# Autodesk Inventor assembly: Complete Device
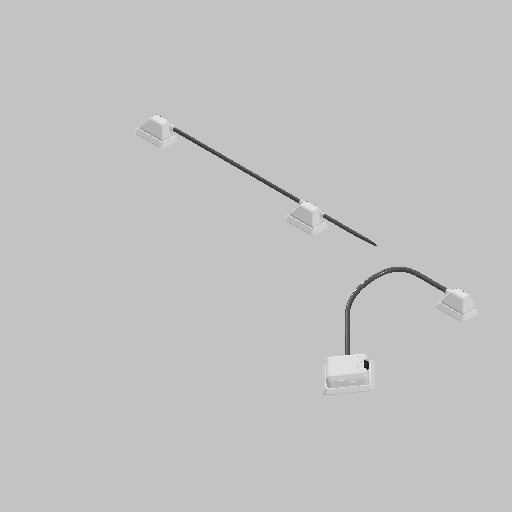
[picture p0: Inventor's stored thumbnail of the model, 512x512]
Saved by Autodesk Inventor 2025.2 (Build 292293000, 293)
## iProperties
Created: 2024-11-20
Part Number: Complete Device
Document SubType Name: Assembly
Designer: tills
Author: tills
## Documents named in this file (8)
- C:\Users\matss\Documents\.Studium\Health_Device\CAD\Wearable-Health-Device\Complete Device.iam
- C:\Users\matss\Documents\.Studium\Health_Device\CAD\Wearable-Health-Device\Inventor_AKTUELL\ASM IMU mitte.iam
- C:\Users\matss\Documents\.Studium\Health_Device\CAD\Wearable-Health-Device\Inventor_AKTUELL\ASM IMU unten.iam
- C:\Users\matss\Documents\.Studium\Health_Device\CAD\Wearable-Health-Device\ASM Main.iam
- C:\Users\matss\Documents\.Studium\Health_Device\CAD\Wearable-Health-Device\kabel.ipt
- C:\Users\matss\Documents\.Studium\Health_Device\CAD\Wearable-Health-Device\Inventor_AKTUELL\ASM IMU oben.iam
- C:\Users\matss\Documents\.Studium\Health_Device\CAD\Wearable-Health-Device\kabel2.ipt
- C:\Users\matss\Documents\.Studium\Health_Device\CAD\Wearable-Health-Device\Kabel3.ipt
## Components (7 placed, 7 different names)
1. ASM IMU mitte:1 [sub-assembly] — Mate:3, Mate:4, Flush:1, Flush:2, Mate:5, Mate:6, Mate:7, Mate:14, Mate:15, Mate:16, Flush:3
2. ASM IMU unten:1 [sub-assembly] — Mate:1, Mate:2, Flush:3, Angle:3
3. ASM Main:1 [sub-assembly] — Mate:11, Mate:12, Angle:2
4. kabel:1 — Mate:1, Mate:2, Mate:3, Mate:4, Angle:3
5. ASM IMU oben:1 [sub-assembly] — Flush:1, Flush:2, Mate:8, Mate:9, Mate:10, Angle:1, Mate:13
6. kabel2:1 — Mate:5, Mate:6, Mate:7, Mate:8, Mate:13
7. Kabel3:1 — Mate:9, Mate:10, Angle:1, Mate:11, Mate:12, Angle:2
## Relationships (22: Mate 16, Flush 3, Angle 3)
- Mate:1: ASM IMU unten:1 ↔ kabel:1
- Mate:2: ASM IMU unten:1 ↔ kabel:1
- Mate:3: ASM IMU mitte:1 ↔ kabel:1
- Mate:4: ASM IMU mitte:1 ↔ kabel:1
- Flush:1: ASM IMU mitte:1 ↔ ASM IMU oben:1
- Flush:2: ASM IMU mitte:1 ↔ ASM IMU oben:1
- Mate:5: ASM IMU mitte:1 ↔ kabel2:1
- Mate:6: ASM IMU mitte:1 ↔ kabel2:1
- Mate:7: ASM IMU mitte:1 ↔ kabel2:1
- Mate:8: ASM IMU oben:1 ↔ kabel2:1
- Mate:9: ASM IMU oben:1 ↔ Kabel3:1
- Mate:10: ASM IMU oben:1 ↔ Kabel3:1
- Angle:1 (-10 deg): ASM IMU oben:1 ↔ Kabel3:1
- Mate:11: ASM Main:1 ↔ Kabel3:1
- Mate:12: ASM Main:1 ↔ Kabel3:1
- Angle:2 (0 deg): ASM Main:1 ↔ Kabel3:1
- Mate:13: ASM IMU oben:1 ↔ kabel2:1
- Mate:14: ASM IMU mitte:1
- Mate:15: ASM IMU mitte:1
- Mate:16: ASM IMU mitte:1
- Flush:3: ASM IMU mitte:1 ↔ ASM IMU unten:1
- Angle:3 (0 deg): ASM IMU unten:1 ↔ kabel:1
